# Autodesk Inventor assembly: AM14U3 Long Frame Half
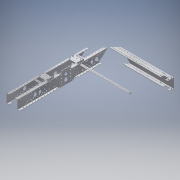
[picture p0: Inventor's stored thumbnail of the model, 180x180]
Saved by Autodesk Inventor 2016 (Build 200138000, 138)
## iProperties
Created: 2016-01-13
Part Number: AM14U3 Long Frame Half
Document SubType Name: Assembly
Designer: Douglas
Author: Douglas
Revision Number: ANY
## Documents named in this file (10)
- D:\Douglas\Documents\Git\2016-Robot-CAD\Inventor\Chassis\AM14U3 Long Frame Half.iam
- D:\Douglas\Documents\Git\2016-Robot-CAD\Inventor\Chassis\Churro 3375.ipt
- D:\Douglas\Documents\Git\2016-Robot-CAD\Inventor\Chassis\FHTS 0.25-20-0.75_FHTS 0.25-20-G-0.75-C.ipt
- D:\Douglas\Documents\Git\2016-Robot-CAD\Inventor\Chassis\Churro 16250.ipt
- D:\Douglas\Documents\Git\2016-Robot-CAD\Inventor\Chassis\10-32x0500_shcs_HX-SHCS 0.19-32x1.375x1-C.ipt
- D:\Douglas\Documents\Git\2016-Robot-CAD\Inventor\Chassis\10-32 Nylock Nut.ipt
- D:\Douglas\Documents\Git\2016-Robot-CAD\Inventor\Chassis\AM14U3 End Sheet Long.ipt
- D:\Douglas\Documents\Git\2016-Robot-CAD\Inventor\Chassis\AM14U3 Inside Sheet Rev2.ipt
- D:\Douglas\Documents\Git\2016-Robot-CAD\Inventor\Chassis\AM14U3 Outside Sheet Rev1_DefaultSM-FLAT-PATTERN.ipt
- D:\Douglas\Documents\Git\2016-Robot-CAD\Inventor\Chassis\am-2954 AM14U2 2x3 Hole Bracket.ipt
## Components (60 placed, 60 different names)
1. Churro 3375_80 — Mate:1, Mate:2, Mate:3, Mate:5
2. Churro 3375_81 — Mate:58, Mate:59, Mate:60, Mate:62
3. Churro 3375_82 — Mate:7, Mate:8, Mate:9, Mate:10
4. Churro 3375_83 — Mate:52, Mate:53, Mate:54, Mate:55
5. FHTS 0.25-20-0.75_FHTS 0.25-20-G-0.75-C_84 — Mate:60, Mate:61
6. FHTS 0.25-20-0.75_FHTS 0.25-20-G-0.75-C_85 — Mate:3, Mate:4
7. FHTS 0.25-20-0.75_FHTS 0.25-20-G-0.75-C_86 — Mate:9, Mate:12
8. FHTS 0.25-20-0.75_FHTS 0.25-20-G-0.75-C_87 — Mate:55, Mate:56
9. FHTS 0.25-20-0.75_FHTS 0.25-20-G-0.75-C_88 — Mate:62, Mate:63
10. FHTS 0.25-20-0.75_FHTS 0.25-20-G-0.75-C_89 — Mate:5, Mate:6
11. FHTS 0.25-20-0.75_FHTS 0.25-20-G-0.75-C_90 — Mate:54, Mate:57
12. FHTS 0.25-20-0.75_FHTS 0.25-20-G-0.75-C_91 — Mate:10, Mate:11
13. FHTS 0.25-20-0.75_FHTS 0.25-20-G-0.75-C_92
14. FHTS 0.25-20-0.75_FHTS 0.25-20-G-0.75-C_93
15. Churro 16250_94
16. 10-32x0500_shcs_HX-SHCS 0.19-32x1.375x1-C_95 — Mate:71, Mate:72, Mate:73
17. 10-32x0500_shcs_HX-SHCS 0.19-32x1.375x1-C_96 — Mate:77, Mate:78, Mate:79
18. 10-32x0500_shcs_HX-SHCS 0.19-32x1.375x1-C_97 — Mate:67, Mate:68, Mate:69
19. 10-32x0500_shcs_HX-SHCS 0.19-32x1.375x1-C_98 — Mate:75, Mate:76, Mate:80
20. 10-32x0500_shcs_HX-SHCS 0.19-32x1.375x1-C_99 — Mate:84, Mate:85, Mate:88
21. 10-32x0500_shcs_HX-SHCS 0.19-32x1.375x1-C_100 — Mate:83, Mate:86, Mate:87
22. 10-32x0500_shcs_HX-SHCS 0.19-32x1.375x1-C_101
23. 10-32x0500_shcs_HX-SHCS 0.19-32x1.375x1-C_102
24. 10-32x0500_shcs_HX-SHCS 0.19-32x1.375x1-C_103
25. 10-32x0500_shcs_HX-SHCS 0.19-32x1.375x1-C_104
26. 10-32x0500_shcs_HX-SHCS 0.19-32x1.375x1-C_105
27. 10-32x0500_shcs_HX-SHCS 0.19-32x1.375x1-C_106
28. 10-32 Nylock Nut_107
29. 10-32 Nylock Nut_108
30. 10-32 Nylock Nut_109
31. 10-32 Nylock Nut_110
32. 10-32 Nylock Nut_111
33. 10-32 Nylock Nut_112
34. 10-32 Nylock Nut_113 — Mate:69, Mate:70
35. 10-32 Nylock Nut_114 — Mate:80, Mate:81
36. 10-32 Nylock Nut_115 — Mate:73, Mate:74
37. 10-32 Nylock Nut_116 — Mate:79, Mate:82
38. 10-32 Nylock Nut_117 — Mate:88, Mate:90
39. 10-32 Nylock Nut_118 — Mate:87, Mate:89
40. 10-32x0500_shcs_HX-SHCS 0.19-32x1.375x1-C_119 — Mate:36, Mate:39, Mate:46
41. 10-32x0500_shcs_HX-SHCS 0.19-32x1.375x1-C_120 — Mate:35, Mate:40, Mate:47
42. 10-32x0500_shcs_HX-SHCS 0.19-32x1.375x1-C_121 — Mate:38, Mate:42, Mate:45
43. 10-32x0500_shcs_HX-SHCS 0.19-32x1.375x1-C_122 — Mate:37, Mate:43, Mate:44
44. 10-32x0500_shcs_HX-SHCS 0.19-32x1.375x1-C_123 — Mate:18, Mate:21, Mate:27
45. 10-32x0500_shcs_HX-SHCS 0.19-32x1.375x1-C_124 — Mate:19, Mate:20, Mate:26
46. 10-32x0500_shcs_HX-SHCS 0.19-32x1.375x1-C_125 — Mate:16, Mate:22, Mate:25
47. 10-32x0500_shcs_HX-SHCS 0.19-32x1.375x1-C_126 — Mate:17, Mate:23, Mate:24
48. 10-32 Nylock Nut_127 — Mate:24, Mate:30
49. 10-32 Nylock Nut_128 — Mate:25, Mate:31
50. 10-32 Nylock Nut_129 — Mate:27, Mate:28
51. 10-32 Nylock Nut_130 — Mate:26, Mate:29
52. 10-32 Nylock Nut_131 — Mate:44, Mate:50
53. 10-32 Nylock Nut_132 — Mate:46, Mate:49
54. 10-32 Nylock Nut_133 — Mate:47, Mate:48
55. 10-32 Nylock Nut_134 — Mate:45, Mate:51
56. AM14U3 End Sheet Long_135 — Mate:64, Mate:65, Mate:66, Mate:67, Mate:70, Mate:71, Mate:74, Mate:81, Mate:82, Mate:83, Mate:89, Mate:90
57. AM14U3 Inside Sheet Rev2_136 — Mate:1, Mate:2, Mate:4, Mate:7, Mate:8, Mate:12, Mate:13, Mate:14, Mate:22, Mate:23, Mate:32, Mate:33, Mate:42, Mate:43, Mate:52, Mate:56, Mate:58, Mate:61, Mate:64, Mate:75, Mate:76, Mate:77, Mate:78, Mate:84, Mate:85
58. AM14U3 Outside Sheet Rev1_DefaultSM-FLAT-PATTERN_137 — Mate:6, Mate:11, Mate:15, Mate:20, Mate:21, Mate:34, Mate:39, Mate:40, Mate:53, Mate:57, Mate:59, Mate:63, Mate:65, Mate:66, Mate:68, Mate:72, Mate:86
59. am-2954 AM14U2 2x3 Hole Bracket_138 — Mate:32, Mate:33, Mate:34, Mate:35, Mate:36, Mate:37, Mate:38, Mate:48, Mate:49, Mate:50, Mate:51
60. am-2954 AM14U2 2x3 Hole Bracket_139 — Mate:13, Mate:14, Mate:15, Mate:16, Mate:17, Mate:18, Mate:19, Mate:28, Mate:29, Mate:30, Mate:31
## Relationships (89: Mate 89)
- Mate:1: Churro 3375_80 ↔ AM14U3 Inside Sheet Rev2_136
- Mate:2: Churro 3375_80 ↔ AM14U3 Inside Sheet Rev2_136
- Mate:3: Churro 3375_80 ↔ FHTS 0.25-20-0.75_FHTS 0.25-20-G-0.75-C_85
- Mate:4: FHTS 0.25-20-0.75_FHTS 0.25-20-G-0.75-C_85 ↔ AM14U3 Inside Sheet Rev2_136
- Mate:5: Churro 3375_80 ↔ FHTS 0.25-20-0.75_FHTS 0.25-20-G-0.75-C_89
- Mate:6: FHTS 0.25-20-0.75_FHTS 0.25-20-G-0.75-C_89 ↔ AM14U3 Outside Sheet Rev1_DefaultSM-FLAT-PATTERN_137
- Mate:7: Churro 3375_82 ↔ AM14U3 Inside Sheet Rev2_136
- Mate:8: Churro 3375_82 ↔ AM14U3 Inside Sheet Rev2_136
- Mate:9: Churro 3375_82 ↔ FHTS 0.25-20-0.75_FHTS 0.25-20-G-0.75-C_86
- Mate:10: Churro 3375_82 ↔ FHTS 0.25-20-0.75_FHTS 0.25-20-G-0.75-C_91
- Mate:11: FHTS 0.25-20-0.75_FHTS 0.25-20-G-0.75-C_91 ↔ AM14U3 Outside Sheet Rev1_DefaultSM-FLAT-PATTERN_137
- Mate:12: FHTS 0.25-20-0.75_FHTS 0.25-20-G-0.75-C_86 ↔ AM14U3 Inside Sheet Rev2_136
- Mate:13: AM14U3 Inside Sheet Rev2_136 ↔ am-2954 AM14U2 2x3 Hole Bracket_139
- Mate:14: AM14U3 Inside Sheet Rev2_136 ↔ am-2954 AM14U2 2x3 Hole Bracket_139
- Mate:15: AM14U3 Outside Sheet Rev1_DefaultSM-FLAT-PATTERN_137 ↔ am-2954 AM14U2 2x3 Hole Bracket_139
- Mate:16: 10-32x0500_shcs_HX-SHCS 0.19-32x1.375x1-C_125 ↔ am-2954 AM14U2 2x3 Hole Bracket_139
- Mate:17: 10-32x0500_shcs_HX-SHCS 0.19-32x1.375x1-C_126 ↔ am-2954 AM14U2 2x3 Hole Bracket_139
- Mate:18: 10-32x0500_shcs_HX-SHCS 0.19-32x1.375x1-C_123 ↔ am-2954 AM14U2 2x3 Hole Bracket_139
- Mate:19: 10-32x0500_shcs_HX-SHCS 0.19-32x1.375x1-C_124 ↔ am-2954 AM14U2 2x3 Hole Bracket_139
- Mate:20: 10-32x0500_shcs_HX-SHCS 0.19-32x1.375x1-C_124 ↔ AM14U3 Outside Sheet Rev1_DefaultSM-FLAT-PATTERN_137
- Mate:21: 10-32x0500_shcs_HX-SHCS 0.19-32x1.375x1-C_123 ↔ AM14U3 Outside Sheet Rev1_DefaultSM-FLAT-PATTERN_137
- Mate:22: 10-32x0500_shcs_HX-SHCS 0.19-32x1.375x1-C_125 ↔ AM14U3 Inside Sheet Rev2_136
- Mate:23: 10-32x0500_shcs_HX-SHCS 0.19-32x1.375x1-C_126 ↔ AM14U3 Inside Sheet Rev2_136
- Mate:24: 10-32x0500_shcs_HX-SHCS 0.19-32x1.375x1-C_126 ↔ 10-32 Nylock Nut_127
- Mate:25: 10-32x0500_shcs_HX-SHCS 0.19-32x1.375x1-C_125 ↔ 10-32 Nylock Nut_128
- Mate:26: 10-32x0500_shcs_HX-SHCS 0.19-32x1.375x1-C_124 ↔ 10-32 Nylock Nut_130
- Mate:27: 10-32x0500_shcs_HX-SHCS 0.19-32x1.375x1-C_123 ↔ 10-32 Nylock Nut_129
- Mate:28: 10-32 Nylock Nut_129 ↔ am-2954 AM14U2 2x3 Hole Bracket_139
- Mate:29: 10-32 Nylock Nut_130 ↔ am-2954 AM14U2 2x3 Hole Bracket_139
- Mate:30: 10-32 Nylock Nut_127 ↔ am-2954 AM14U2 2x3 Hole Bracket_139
- Mate:31: 10-32 Nylock Nut_128 ↔ am-2954 AM14U2 2x3 Hole Bracket_139
- Mate:32: AM14U3 Inside Sheet Rev2_136 ↔ am-2954 AM14U2 2x3 Hole Bracket_138
- Mate:33: AM14U3 Inside Sheet Rev2_136 ↔ am-2954 AM14U2 2x3 Hole Bracket_138
- Mate:34: AM14U3 Outside Sheet Rev1_DefaultSM-FLAT-PATTERN_137 ↔ am-2954 AM14U2 2x3 Hole Bracket_138
- Mate:35: 10-32x0500_shcs_HX-SHCS 0.19-32x1.375x1-C_120 ↔ am-2954 AM14U2 2x3 Hole Bracket_138
- Mate:36: 10-32x0500_shcs_HX-SHCS 0.19-32x1.375x1-C_119 ↔ am-2954 AM14U2 2x3 Hole Bracket_138
- Mate:37: 10-32x0500_shcs_HX-SHCS 0.19-32x1.375x1-C_122 ↔ am-2954 AM14U2 2x3 Hole Bracket_138
- Mate:38: 10-32x0500_shcs_HX-SHCS 0.19-32x1.375x1-C_121 ↔ am-2954 AM14U2 2x3 Hole Bracket_138
- Mate:39: 10-32x0500_shcs_HX-SHCS 0.19-32x1.375x1-C_119 ↔ AM14U3 Outside Sheet Rev1_DefaultSM-FLAT-PATTERN_137
- Mate:40: 10-32x0500_shcs_HX-SHCS 0.19-32x1.375x1-C_120 ↔ AM14U3 Outside Sheet Rev1_DefaultSM-FLAT-PATTERN_137
- Mate:42: 10-32x0500_shcs_HX-SHCS 0.19-32x1.375x1-C_121 ↔ AM14U3 Inside Sheet Rev2_136
- Mate:43: 10-32x0500_shcs_HX-SHCS 0.19-32x1.375x1-C_122 ↔ AM14U3 Inside Sheet Rev2_136
- Mate:44: 10-32x0500_shcs_HX-SHCS 0.19-32x1.375x1-C_122 ↔ 10-32 Nylock Nut_131
- Mate:45: 10-32x0500_shcs_HX-SHCS 0.19-32x1.375x1-C_121 ↔ 10-32 Nylock Nut_134
- Mate:46: 10-32x0500_shcs_HX-SHCS 0.19-32x1.375x1-C_119 ↔ 10-32 Nylock Nut_132
- Mate:47: 10-32x0500_shcs_HX-SHCS 0.19-32x1.375x1-C_120 ↔ 10-32 Nylock Nut_133
- Mate:48: 10-32 Nylock Nut_133 ↔ am-2954 AM14U2 2x3 Hole Bracket_138
- Mate:49: 10-32 Nylock Nut_132 ↔ am-2954 AM14U2 2x3 Hole Bracket_138
- Mate:50: 10-32 Nylock Nut_131 ↔ am-2954 AM14U2 2x3 Hole Bracket_138
- Mate:51: 10-32 Nylock Nut_134 ↔ am-2954 AM14U2 2x3 Hole Bracket_138
- Mate:52: Churro 3375_83 ↔ AM14U3 Inside Sheet Rev2_136
- Mate:53: Churro 3375_83 ↔ AM14U3 Outside Sheet Rev1_DefaultSM-FLAT-PATTERN_137
- Mate:54: Churro 3375_83 ↔ FHTS 0.25-20-0.75_FHTS 0.25-20-G-0.75-C_90
- Mate:55: Churro 3375_83 ↔ FHTS 0.25-20-0.75_FHTS 0.25-20-G-0.75-C_87
- Mate:56: FHTS 0.25-20-0.75_FHTS 0.25-20-G-0.75-C_87 ↔ AM14U3 Inside Sheet Rev2_136
- Mate:57: FHTS 0.25-20-0.75_FHTS 0.25-20-G-0.75-C_90 ↔ AM14U3 Outside Sheet Rev1_DefaultSM-FLAT-PATTERN_137
- Mate:58: Churro 3375_81 ↔ AM14U3 Inside Sheet Rev2_136
- Mate:59: Churro 3375_81 ↔ AM14U3 Outside Sheet Rev1_DefaultSM-FLAT-PATTERN_137
- Mate:60: Churro 3375_81 ↔ FHTS 0.25-20-0.75_FHTS 0.25-20-G-0.75-C_84
- Mate:61: FHTS 0.25-20-0.75_FHTS 0.25-20-G-0.75-C_84 ↔ AM14U3 Inside Sheet Rev2_136
- Mate:62: Churro 3375_81 ↔ FHTS 0.25-20-0.75_FHTS 0.25-20-G-0.75-C_88
- Mate:63: FHTS 0.25-20-0.75_FHTS 0.25-20-G-0.75-C_88 ↔ AM14U3 Outside Sheet Rev1_DefaultSM-FLAT-PATTERN_137
- Mate:64: AM14U3 End Sheet Long_135 ↔ AM14U3 Inside Sheet Rev2_136
- Mate:65: AM14U3 End Sheet Long_135 ↔ AM14U3 Outside Sheet Rev1_DefaultSM-FLAT-PATTERN_137
- Mate:66: AM14U3 End Sheet Long_135 ↔ AM14U3 Outside Sheet Rev1_DefaultSM-FLAT-PATTERN_137
- Mate:67: 10-32x0500_shcs_HX-SHCS 0.19-32x1.375x1-C_97 ↔ AM14U3 End Sheet Long_135
- Mate:68: 10-32x0500_shcs_HX-SHCS 0.19-32x1.375x1-C_97 ↔ AM14U3 Outside Sheet Rev1_DefaultSM-FLAT-PATTERN_137
- Mate:69: 10-32x0500_shcs_HX-SHCS 0.19-32x1.375x1-C_97 ↔ 10-32 Nylock Nut_113
- Mate:70: 10-32 Nylock Nut_113 ↔ AM14U3 End Sheet Long_135
- Mate:71: 10-32x0500_shcs_HX-SHCS 0.19-32x1.375x1-C_95 ↔ AM14U3 End Sheet Long_135
- Mate:72: 10-32x0500_shcs_HX-SHCS 0.19-32x1.375x1-C_95 ↔ AM14U3 Outside Sheet Rev1_DefaultSM-FLAT-PATTERN_137
- Mate:73: 10-32x0500_shcs_HX-SHCS 0.19-32x1.375x1-C_95 ↔ 10-32 Nylock Nut_115
- Mate:74: 10-32 Nylock Nut_115 ↔ AM14U3 End Sheet Long_135
- Mate:75: 10-32x0500_shcs_HX-SHCS 0.19-32x1.375x1-C_98 ↔ AM14U3 Inside Sheet Rev2_136
- Mate:76: 10-32x0500_shcs_HX-SHCS 0.19-32x1.375x1-C_98 ↔ AM14U3 Inside Sheet Rev2_136
- Mate:77: 10-32x0500_shcs_HX-SHCS 0.19-32x1.375x1-C_96 ↔ AM14U3 Inside Sheet Rev2_136
- Mate:78: 10-32x0500_shcs_HX-SHCS 0.19-32x1.375x1-C_96 ↔ AM14U3 Inside Sheet Rev2_136
- Mate:79: 10-32x0500_shcs_HX-SHCS 0.19-32x1.375x1-C_96 ↔ 10-32 Nylock Nut_116
- Mate:80: 10-32x0500_shcs_HX-SHCS 0.19-32x1.375x1-C_98 ↔ 10-32 Nylock Nut_114
- Mate:81: 10-32 Nylock Nut_114 ↔ AM14U3 End Sheet Long_135
- Mate:82: 10-32 Nylock Nut_116 ↔ AM14U3 End Sheet Long_135
- Mate:83: 10-32x0500_shcs_HX-SHCS 0.19-32x1.375x1-C_100 ↔ AM14U3 End Sheet Long_135
- Mate:84: 10-32x0500_shcs_HX-SHCS 0.19-32x1.375x1-C_99 ↔ AM14U3 Inside Sheet Rev2_136
- Mate:85: 10-32x0500_shcs_HX-SHCS 0.19-32x1.375x1-C_99 ↔ AM14U3 Inside Sheet Rev2_136
- Mate:86: 10-32x0500_shcs_HX-SHCS 0.19-32x1.375x1-C_100 ↔ AM14U3 Outside Sheet Rev1_DefaultSM-FLAT-PATTERN_137
- Mate:87: 10-32x0500_shcs_HX-SHCS 0.19-32x1.375x1-C_100 ↔ 10-32 Nylock Nut_118
- Mate:88: 10-32x0500_shcs_HX-SHCS 0.19-32x1.375x1-C_99 ↔ 10-32 Nylock Nut_117
- Mate:89: 10-32 Nylock Nut_118 ↔ AM14U3 End Sheet Long_135
- Mate:90: 10-32 Nylock Nut_117 ↔ AM14U3 End Sheet Long_135
